# Autodesk Inventor assembly: drivetrain
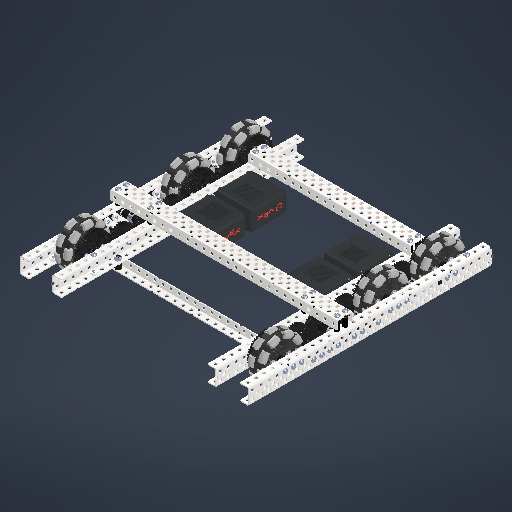
[picture p0: Inventor's stored thumbnail of the model, 512x512]
Saved by Autodesk Inventor 2026.1 (Build 301233000, 233)
## iProperties
Created: 2024-09-29
Part Number: drivetrain
Document SubType Name: Assembly
Designer: Exortions
Author: Exortions
## Documents named in this file (34)
- C:\Users\shimo\OneDrive\Documents\GitHub\cad3284b-2024\second-robot\drivetrain - Copy.iam
- C:\Users\shimo\OneDrive\Documents\GitHub\cad3284b-2024\lib\vex\Structure\C Channel\Aluminum 1x2x1\Alu C 1x2x1x30.ipt
- C:\Users\shimo\OneDrive\Documents\GitHub\cad3284b-2024\lib\vex\Structure\C Channel\Aluminum 1x2x1\Alu C 1x2x1x28.ipt
- C:\Users\shimo\OneDrive\Documents\GitHub\cad3284b-2024\lib\vex\Structure\Hardware\Screw Steel - Star\SScrew Star Smooth .290.ipt
- C:\Users\shimo\OneDrive\Documents\GitHub\cad3284b-2024\lib\vex\Structure\Standoff\Standoff .75.ipt
- C:\Users\shimo\OneDrive\Documents\GitHub\cad3284b-2024\lib\vex\Structure\C Channel\Aluminum 1x2x1\Alu C 1x2x1x26.ipt
- C:\Users\shimo\OneDrive\Documents\GitHub\cad3284b-2024\lib\vex\Structure\C Channel\Aluminum 1x2x1\Alu C 1x2x1x20.ipt
- C:\Users\shimo\OneDrive\Documents\GitHub\cad3284b-2024\lib\vex\Motion\Spacers\Spacer Nylon .375 OD\NSpacer .375 OD x .500.ipt
- C:\Users\shimo\OneDrive\Documents\GitHub\cad3284b-2024\lib\vex\Motion\Spacers\Spacer Nylon .375 OD\NSpacer .375 OD x .375.ipt
- C:\Users\shimo\OneDrive\Documents\GitHub\cad3284b-2024\lib\vex\Structure\Hardware\Nut Alu.ipt
- C:\Users\shimo\OneDrive\Documents\GitHub\cad3284b-2024\lib\vex\Structure\Hardware\Nut Thin Nylock.ipt
- C:\Users\shimo\OneDrive\Documents\GitHub\cad3284b-2024\lib\vex\Structure\Hardware\Screw Steel - Star\SScrew Star Smooth 2.250.ipt
- C:\Users\shimo\OneDrive\Documents\GitHub\cad3284b-2024\second-robot\drivetrain-wheel.iam
- C:\Users\shimo\OneDrive\Documents\GitHub\cad3284b-2024\lib\vex\Structure\Hardware\Nut Keps.ipt
- C:\Users\shimo\OneDrive\Documents\GitHub\cad3284b-2024\lib\vex\Motion\Shaft LS\Bearing Flat.ipt
- C:\Users\shimo\OneDrive\Documents\GitHub\cad3284b-2024\lib\vex\Structure\Hardware\Screw Steel - Star\SScrew Star Smooth .500.ipt
- C:\Users\shimo\OneDrive\Documents\GitHub\cad3284b-2024\lib\vex\Structure\Hardware\Nut Nylon\Nut Nylon - White.ipt
- C:\Users\shimo\OneDrive\Documents\GitHub\cad3284b-2024\lib\vex\Electronics\V5 Motor.ipt
- C:\Users\shimo\OneDrive\Documents\GitHub\cad3284b-2024\lib\vex\Motion\Gears\LS 36T Gear.ipt
- C:\Users\shimo\OneDrive\Documents\GitHub\cad3284b-2024\lib\vex\Motion\Spacers\Washer Teflon\TWasher .375 OD x .06250.ipt
- C:\Users\shimo\OneDrive\Documents\GitHub\cad3284b-2024\lib\vex\Motion\Shaft LS\Shaft Collar ipts\Shaft Collar Set Screw.ipt
- C:\Users\shimo\OneDrive\Documents\GitHub\cad3284b-2024\lib\vex\Motion\Spacers\Spacer Nylon .375 OD\NSpacer .375 OD x .125.ipt
- C:\Users\shimo\OneDrive\Documents\GitHub\cad3284b-2024\lib\vex\Motion\1-Post Bearing Flat Hex Retainer.ipt
- C:\Users\shimo\OneDrive\Documents\GitHub\cad3284b-2024\lib\vex\Structure\C Channel\Aluminum 1x2x1\Alu C 1x2x1x1.ipt
- C:\Users\shimo\OneDrive\Documents\GitHub\cad3284b-2024\lib\vex\Structure\Angle\Aluminum 1x1\Alu Angle 1x1x20.ipt
- C:\Users\shimo\OneDrive\Documents\GitHub\cad3284b-2024\lib\vex\Structure\Hardware\Screw Steel - Star\SScrew Star Smooth .625.ipt
- C:\Users\shimo\OneDrive\Documents\GitHub\cad3284b-2024\lib\vex\Structure\Hardware\Screw Steel - Star.ipt
- C:\Users\shimo\OneDrive\Documents\GitHub\cad3284b-2024\lib\vex\Structure\Standoff.ipt
- C:\Users\shimo\OneDrive\Documents\GitHub\cad3284b-2024\lib\vex\Structure\Hardware\Nut Nylon.ipt
- C:\Users\shimo\OneDrive\Documents\GitHub\cad3284b-2024\lib\vex\Motion\Spacers\Washer Teflon.ipt
- C:\Users\shimo\OneDrive\Documents\GitHub\cad3284b-2024\lib\vex\Motion\Spacers\Spacer Nylon .375 OD.ipt
- C:\Users\shimo\OneDrive\Documents\GitHub\cad3284b-2024\lib\vex\Structure\Standoff\Standoff .50.ipt
- C:\Users\shimo\OneDrive\Documents\GitHub\3284b-highlander-cad\Library\VEX-CAD-Inventor-1.4.2\Structure\C Channel\Aluminum 1x2x1\Alu C 1x2x1x2.ipt
- C:\Users\shimo\OneDrive\Documents\GitHub\3284b-highlander-cad\Library\VEX-CAD-Inventor-1.4.2\Structure\C Channel\Aluminum 1x2x1\Alu C 1x2x1x1.ipt
## Components (224 placed, 27 different names)
1. Alu C 1x2x1x30:1 — Insert:1, Insert:2, Insert:5, Insert:6, Insert:13, Insert:14, Insert:66, Insert:69, Insert:70, Insert:72, Insert:73, Insert:78, Insert:79, Insert:80, Insert:81, Insert:223, Insert:224, Insert:228, Insert:229, Insert:232, Insert:233, Insert:238, Insert:239, Insert:245, Insert:246, Insert:247, Insert:248, Insert:249, Insert:250, Insert:251, Insert:253, Insert:254, Insert:255, Insert:256, Insert:267, Insert:268, Insert:270, Insert:271, Insert:275, Insert:455, Insert:1085
2. Alu C 1x2x1x30:2 — Insert:3, Insert:4, Insert:11, Insert:12, Insert:15, Insert:16, Insert:293, Insert:294, Insert:295, Insert:296, Insert:297, Insert:301, Insert:302, Insert:303, Insert:304, Insert:305, Insert:335, Insert:336, Insert:341, Insert:342, Insert:343, Insert:344, Insert:345, Insert:346, Insert:347, Insert:348, Insert:349, Insert:350, Insert:377, Insert:378, Insert:379, Insert:380, Insert:408, Insert:433, Insert:473
3. Alu C 1x2x1x28:1 — Insert:1, Insert:2, Insert:3, Insert:4, Insert:7, Insert:8, Insert:9, Insert:10, Insert:17, Insert:18, Insert:19, Insert:20, Insert:25, Insert:26, Insert:31, Insert:32, Insert:506, Insert:507, Insert:532, Insert:533, Insert:534, Insert:535
4. SScrew Star Smooth .290:1 — Insert:8
5. SScrew Star Smooth .290:2 — Insert:6
6. SScrew Star Smooth .290:3 — Insert:7
7. SScrew Star Smooth .290:4 — Insert:5
8. SScrew Star Smooth .290:5 — Insert:12
9. SScrew Star Smooth .290:6 — Insert:10
10. SScrew Star Smooth .290:7 — Insert:9
11. SScrew Star Smooth .290:8 — Insert:11
12. Standoff .75:1 — Insert:14
13. Standoff .75:2 — Insert:13
14. Standoff .75:3 — Insert:16
15. Standoff .75:4 — Insert:15
16. Alu C 1x2x1x26:1 — Insert:25, Insert:26, Insert:27, Insert:28, Insert:29, Insert:30, Insert:44, Insert:193, Insert:225, Insert:226, Mate:2, Flush:3, Flush:4, Insert:240, Insert:244, Insert:257, Insert:264, Insert:266, Insert:276, Insert:453, Insert:454, Insert:482, Insert:483, Insert:484, Insert:485, Insert:490, Insert:520, Insert:521, Insert:522, Insert:523, Insert:698, Insert:699, Insert:702, Insert:1034, Insert:1055, Insert:1056, Rigid:4
17. Alu C 1x2x1x26:2 — Insert:19, Insert:20, Insert:21, Insert:22, Insert:23, Insert:24, Insert:46, Mate:1, Flush:1, Flush:2, Insert:325, Insert:327, Insert:331, Insert:332, Insert:369, Insert:375, Insert:409, Insert:431, Insert:432, Insert:451, Insert:475, Insert:476, Insert:479, Insert:480, Insert:481, Insert:491, Insert:512, Insert:513, Insert:514, Insert:515, Insert:704, Insert:1036, Insert:1053, Insert:1054, Rigid:3
18. SScrew Star Smooth .290:9 — Insert:18
19. SScrew Star Smooth .290:10 — Insert:17
20. Standoff .75:5 — Insert:21
21. Standoff .75:6 — Insert:22
22. SScrew Star Smooth .290:11 — Insert:32
23. SScrew Star Smooth .290:12 — Insert:31
24. Standoff .75:7 — Insert:30
25. Standoff .75:8 — Insert:29
26. SScrew Star Smooth .290:13 — Insert:24
27. SScrew Star Smooth .290:14 — Insert:23
28. SScrew Star Smooth .290:15 — Insert:28
29. SScrew Star Smooth .290:16 — Insert:27
30. Alu C 1x2x1x20:1 — Insert:36, Insert:37, Insert:38, Insert:39, Insert:698, Insert:699
31. SScrew Star Smooth .290:17 — Insert:36
32. SScrew Star Smooth .290:18 — Insert:37
33. SScrew Star Smooth .290:19 — Insert:38
34. SScrew Star Smooth .290:20 — Insert:39
35. SScrew Star Smooth .290:22 — Insert:44
36. SScrew Star Smooth .290:24 — Insert:46
37. SScrew Star Smooth 2.250:29 — Insert:66
38. Nut Keps:1 — Insert:71
39. Bearing Flat:1 — Insert:69, Insert:70, Insert:71, Insert:74, Insert:75
40. SScrew Star Smooth .500:30 — Insert:73
41. SScrew Star Smooth .500:31 — Insert:72
42. Nut Nylon - White:1 — Insert:75
43. Nut Nylon - White:2 — Insert:74
44. Bearing Flat:2 — Insert:78, Insert:79, Insert:452
45. Nut Nylon - White:3
46. Nut Nylon - White:4
47. SScrew Star Smooth .500:32 — Insert:81
48. SScrew Star Smooth .500:33 — Insert:80
49. LS 36T Gear:1 — Insert:94, Insert:96
50. TWasher .375 OD x .06250:1 — Insert:94, Insert:453
51. NSpacer .375 OD x .500:11 — Insert:96, Insert:97
52. Shaft Collar Set Screw:1 — Insert:97, Insert:99
53. NSpacer .375 OD x .375:12 — Insert:98, Insert:99
54. TWasher .375 OD x .06250:2 — Insert:98
55. Nut Keps:2
56. Bearing Flat:4 — Insert:247, Insert:248
57. Nut Nylon - White:6
58. Nut Nylon - White:7
59. Bearing Flat:6 — Insert:228, Insert:229
60. Nut Nylon - White:10
61. Nut Nylon - White:11
62. NSpacer .375 OD x .125:13 — Insert:234, Insert:454
63. Nut Keps:5 — Insert:269
64. LS 36T Gear:2
65. TWasher .375 OD x .06250:5 — Insert:244
66. NSpacer .375 OD x .500:16
67. Shaft Collar Set Screw:2
68. NSpacer .375 OD x .375:17
69. TWasher .375 OD x .06250:6
70. LS 36T Gear:3
71. TWasher .375 OD x .06250:7 — Insert:264
72. NSpacer .375 OD x .500:18
73. Shaft Collar Set Screw:3
74. NSpacer .375 OD x .375:19
75. TWasher .375 OD x .06250:8
76. Bearing Flat:10 — Insert:238, Insert:239
77. Nut Nylon - White:18
78. Nut Nylon - White:19
79. Bearing Flat:11 — Insert:253, Insert:254
80. Nut Nylon - White:20
81. Nut Nylon - White:21
82. 1-Post Bearing Flat Hex Retainer:1 — Insert:182, Insert:267, Insert:268, Insert:269
83. Nut Nylon - White:22 — Insert:182
84. SScrew Star Smooth .500:62 — Insert:193
85. SScrew Star Smooth .290:67
86. SScrew Star Smooth .290:69
87. SScrew Star Smooth .290:70
88. Nut Nylon - White:25 — Insert:226
89. Nut Nylon - White:26 — Insert:225
90. Nut Nylon - White:27 — Insert:224
91. Nut Nylon - White:28 — Insert:223
92. Alu C 1x2x1x1:1 — Mate:1, Flush:1, Flush:2, Rigid:1
93. Alu C 1x2x1x1:2 — Mate:2, Flush:3, Flush:4, Rigid:2
94. SScrew Star Smooth .500:72 — Insert:232
95. SScrew Star Smooth .500:73 — Insert:233
96. LS 36T Gear:4 — Insert:234, Insert:237
97. NSpacer .375 OD x .500:31 — Insert:236
98. NSpacer .375 OD x .500:32 — Insert:236, Insert:237
99. SScrew Star Smooth .500:74 — Insert:245
100. SScrew Star Smooth .500:75 — Insert:246
101. SScrew Star Smooth .500:76 — Insert:240
102. SScrew Star Smooth .500:77 — Insert:249
103. SScrew Star Smooth 2.250:78 — Insert:250
104. SScrew Star Smooth .500:79 — Insert:251
105. SScrew Star Smooth .500:80 — Insert:256
106. SScrew Star Smooth .500:81 — Insert:255
107. SScrew Star Smooth .500:82 — Insert:257
108. SScrew Star Smooth .500:84 — Insert:266
109. SScrew Star Smooth .500:85 — Insert:270
110. SScrew Star Smooth 2.250:86 — Insert:271
111. SScrew Star Smooth .290:89
112. Nut Nylon - White:31 — Insert:276
113. SScrew Star Smooth .290:90
114. Nut Nylon - White:32 — Insert:275
115. SScrew Star Smooth 2.250:93 — Insert:295
116. Nut Keps:6
117. Bearing Flat:12 — Insert:293, Insert:294
118. SScrew Star Smooth .500:94 — Insert:297
119. SScrew Star Smooth .500:95 — Insert:296
120. Nut Nylon - White:33
121. Nut Nylon - White:34
122. SScrew Star Smooth 2.250:96 — Insert:305
123. Nut Keps:7
124. Bearing Flat:13 — Insert:301, Insert:302
125. SScrew Star Smooth .500:97 — Insert:303
126. SScrew Star Smooth .500:98 — Insert:304
127. Nut Nylon - White:35
128. Nut Nylon - White:36
129. Nut Keps:9
130. 1-Post Bearing Flat Hex Retainer:2 — Insert:377, Insert:378
131. Nut Nylon - White:39
132. SScrew Star Smooth .500:104 — Insert:325
133. SScrew Star Smooth .500:106 — Insert:327
134. SScrew Star Smooth .500:107 — Insert:331
135. SScrew Star Smooth .500:108 — Insert:332
136. Bearing Flat:16 — Insert:335, Insert:336
137. Nut Nylon - White:41
138. Nut Nylon - White:42
139. SScrew Star Smooth .500:109 — Insert:345
140. SScrew Star Smooth .500:110 — Insert:346
141. Bearing Flat:17 — Insert:341, Insert:342
142. Nut Nylon - White:43
143. Nut Nylon - White:44
144. Bearing Flat:18 — Insert:343, Insert:344, Insert:474
145. Nut Nylon - White:45
146. Nut Nylon - White:46
147. SScrew Star Smooth .500:111 — Insert:347
148. SScrew Star Smooth .500:112 — Insert:348
149. SScrew Star Smooth .500:113 — Insert:349
150. SScrew Star Smooth .500:114 — Insert:350
151. NSpacer .375 OD x .125:45 — Insert:475
152. LS 36T Gear:5
153. NSpacer .375 OD x .500:46
154. NSpacer .375 OD x .500:47
155. LS 36T Gear:6
156. TWasher .375 OD x .06250:9 — Insert:476
157. NSpacer .375 OD x .500:48
158. Shaft Collar Set Screw:4
159. NSpacer .375 OD x .375:49
160. TWasher .375 OD x .06250:10
161. LS 36T Gear:7
162. TWasher .375 OD x .06250:11 — Insert:369
163. NSpacer .375 OD x .500:50
164. Shaft Collar Set Screw:5
165. NSpacer .375 OD x .375:51
166. TWasher .375 OD x .06250:12
167. LS 36T Gear:8
168. TWasher .375 OD x .06250:13 — Insert:375
169. NSpacer .375 OD x .500:52
170. Shaft Collar Set Screw:6
171. NSpacer .375 OD x .375:53
172. TWasher .375 OD x .06250:14
173. SScrew Star Smooth .500:116 — Insert:380
174. SScrew Star Smooth 2.250:117 — Insert:379
175. Nut Nylon - White:47 — Insert:408
176. SScrew Star Smooth .290:124
177. SScrew Star Smooth .290:125
178. Nut Nylon - White:48 — Insert:409
179. SScrew Star Smooth .290:130
180. Nut Nylon - White:50 — Insert:433
181. Nut Nylon - White:51 — Insert:432
182. Nut Nylon - White:53 — Insert:431
183. Alu Angle 1x1x20:1 — Insert:451, Insert:485, Insert:486, Insert:487, Insert:488, Insert:489
184. SScrew Star Smooth 2.250:136 — Insert:455
185. Nut Keps:11 — Insert:452
186. SScrew Star Smooth 2.250:140 — Insert:473
187. Nut Keps:12 — Insert:474
188. drivetrain-wheel:1 [sub-assembly] — Insert:479
189. drivetrain-wheel:2 [sub-assembly] — Insert:480
190. drivetrain-wheel:3 [sub-assembly] — Insert:481
191. drivetrain-wheel:4 [sub-assembly] — Insert:484
192. drivetrain-wheel:5 [sub-assembly] — Insert:483
193. drivetrain-wheel:6 [sub-assembly] — Insert:482
194. NSpacer .375 OD x .375:73 — Insert:487
195. NSpacer .375 OD x .375:74 — Insert:486
196. SScrew Star Smooth .625:144 — Insert:489
197. SScrew Star Smooth .625:145 — Insert:488
198. Nut Thin Nylock:11 — Insert:490
199. Nut Thin Nylock:12 — Insert:491
200. Nut Alu:5 — Insert:507
201. Nut Alu:6 — Insert:506
202. V5 Motor:9 — Insert:512, Insert:513
203. V5 Motor:10 — Insert:514, Insert:515
204. V5 Motor:12 — Insert:520, Insert:521
205. V5 Motor:13 — Insert:522, Insert:523
206. Nut Alu:7 — Insert:532
207. Nut Alu:8 — Insert:533
208. Nut Alu:9 — Insert:534
209. Nut Alu:10 — Insert:535
210. SScrew Star Smooth .290:200 — Insert:702
211. SScrew Star Smooth .290:201 — Insert:704
212. Nut Nylon - White:69 — Insert:1034
213. SScrew Star Smooth .290:281
214. Nut Nylon - White:70 — Insert:1036
215. SScrew Star Smooth .290:282
216. Standoff .50:44 — Insert:1055
217. Standoff .50:45 — Insert:1056
218. Standoff .50:46 — Insert:1054
219. Standoff .50:47 — Insert:1053
220. Nut Thin Nylock:56 — Insert:1085
221. Alu C 1x2x1x2:1 — Rigid:4
222. Alu C 1x2x1x2:2 — Rigid:3
223. Alu C 1x2x1x1:4 — Rigid:1
224. Alu C 1x2x1x1:5 — Rigid:2
## Relationships (240: Insert 230, Flush 4, WeldJoint 4, Mate 2)
- Insert:1 (19.05 mm): Alu C 1x2x1x30:1 ↔ Alu C 1x2x1x28:1
- Insert:2 (19.05 mm): Alu C 1x2x1x30:1 ↔ Alu C 1x2x1x28:1
- Insert:3 (19.05 mm): Alu C 1x2x1x30:2 ↔ Alu C 1x2x1x28:1
- Insert:4 (19.05 mm): Alu C 1x2x1x30:2 ↔ Alu C 1x2x1x28:1
- Insert:5: Alu C 1x2x1x30:1 ↔ SScrew Star Smooth .290:4
- Insert:6: Alu C 1x2x1x30:1 ↔ SScrew Star Smooth .290:2
- Insert:7: Alu C 1x2x1x28:1 ↔ SScrew Star Smooth .290:3
- Insert:8: Alu C 1x2x1x28:1 ↔ SScrew Star Smooth .290:1
- Insert:9: Alu C 1x2x1x28:1 ↔ SScrew Star Smooth .290:7
- Insert:10: Alu C 1x2x1x28:1 ↔ SScrew Star Smooth .290:6
- Insert:11: Alu C 1x2x1x30:2 ↔ SScrew Star Smooth .290:8
- Insert:12: Alu C 1x2x1x30:2 ↔ SScrew Star Smooth .290:5
- Insert:13: Alu C 1x2x1x30:1 ↔ Standoff .75:2
- Insert:14: Alu C 1x2x1x30:1 ↔ Standoff .75:1
- Insert:15: Alu C 1x2x1x30:2 ↔ Standoff .75:4
- Insert:16: Alu C 1x2x1x30:2 ↔ Standoff .75:3
- Insert:17: Alu C 1x2x1x28:1 ↔ SScrew Star Smooth .290:10
- Insert:18: Alu C 1x2x1x28:1 ↔ SScrew Star Smooth .290:9
- Insert:19 (19.05 mm): Alu C 1x2x1x28:1 ↔ Alu C 1x2x1x26:2
- Insert:20 (19.05 mm): Alu C 1x2x1x28:1 ↔ Alu C 1x2x1x26:2
- Insert:21: Alu C 1x2x1x26:2 ↔ Standoff .75:5
- Insert:22: Alu C 1x2x1x26:2 ↔ Standoff .75:6
- Insert:23: Alu C 1x2x1x26:2 ↔ SScrew Star Smooth .290:14
- Insert:24: Alu C 1x2x1x26:2 ↔ SScrew Star Smooth .290:13
- Insert:25 (19.05 mm): Alu C 1x2x1x28:1 ↔ Alu C 1x2x1x26:1
- Insert:26 (19.05 mm): Alu C 1x2x1x28:1 ↔ Alu C 1x2x1x26:1
- Insert:27: Alu C 1x2x1x26:1 ↔ SScrew Star Smooth .290:16
- Insert:28: Alu C 1x2x1x26:1 ↔ SScrew Star Smooth .290:15
- Insert:29: Alu C 1x2x1x26:1 ↔ Standoff .75:8
- Insert:30: Alu C 1x2x1x26:1 ↔ Standoff .75:7
- Insert:31: Alu C 1x2x1x28:1 ↔ SScrew Star Smooth .290:12
- Insert:32: Alu C 1x2x1x28:1 ↔ SScrew Star Smooth .290:11
- Insert:36: Alu C 1x2x1x20:1 ↔ SScrew Star Smooth .290:17
- Insert:37: Alu C 1x2x1x20:1 ↔ SScrew Star Smooth .290:18
- Insert:38: Alu C 1x2x1x20:1 ↔ SScrew Star Smooth .290:19
- Insert:39: Alu C 1x2x1x20:1 ↔ SScrew Star Smooth .290:20
- Insert:44: Alu C 1x2x1x26:1 ↔ SScrew Star Smooth .290:22
- Insert:46: Alu C 1x2x1x26:2 ↔ SScrew Star Smooth .290:24
- Insert:66: Alu C 1x2x1x30:1 ↔ SScrew Star Smooth 2.250:29
- Insert:69: Alu C 1x2x1x30:1 ↔ Bearing Flat:1
- Insert:70: Alu C 1x2x1x30:1 ↔ Bearing Flat:1
- Insert:71: Nut Keps:1 ↔ Bearing Flat:1
- Insert:72: Alu C 1x2x1x30:1 ↔ SScrew Star Smooth .500:31
- Insert:73: Alu C 1x2x1x30:1 ↔ SScrew Star Smooth .500:30
- Insert:74: Bearing Flat:1 ↔ Nut Nylon - White:2
- Insert:75: Bearing Flat:1 ↔ Nut Nylon - White:1
- [Insert]: Bearing Flat:2 ↔ Nut Nylon - White:4
- [Insert]: Bearing Flat:2 ↔ Nut Nylon - White:3
- Insert:78: Alu C 1x2x1x30:1 ↔ Bearing Flat:2
- Insert:79: Alu C 1x2x1x30:1 ↔ Bearing Flat:2
- Insert:80: Alu C 1x2x1x30:1 ↔ SScrew Star Smooth .500:33
- Insert:81: Alu C 1x2x1x30:1 ↔ SScrew Star Smooth .500:32
- Insert:94: LS 36T Gear:1 ↔ TWasher .375 OD x .06250:1
- Insert:96: LS 36T Gear:1 ↔ NSpacer .375 OD x .500:11
- Insert:97: NSpacer .375 OD x .500:11 ↔ Shaft Collar Set Screw:1
- Insert:98: NSpacer .375 OD x .375:12 ↔ TWasher .375 OD x .06250:2
- Insert:99: Shaft Collar Set Screw:1 ↔ NSpacer .375 OD x .375:12
- [Insert]: Nut Keps:2 ↔ Bearing Flat:4
- [Insert]: Bearing Flat:4 ↔ Nut Nylon - White:7
- [Insert]: Bearing Flat:4 ↔ Nut Nylon - White:6
- [Insert]: Bearing Flat:6 ↔ Nut Nylon - White:11
- [Insert]: Bearing Flat:6 ↔ Nut Nylon - White:10
- [Insert]: LS 36T Gear:2 ↔ TWasher .375 OD x .06250:5
- [Insert]: LS 36T Gear:2 ↔ NSpacer .375 OD x .500:16
- [Insert]: NSpacer .375 OD x .500:16 ↔ Shaft Collar Set Screw:2
- [Insert]: NSpacer .375 OD x .375:17 ↔ TWasher .375 OD x .06250:6
- [Insert]: Shaft Collar Set Screw:2 ↔ NSpacer .375 OD x .375:17
- [Insert]: LS 36T Gear:3 ↔ TWasher .375 OD x .06250:7
- [Insert]: LS 36T Gear:3 ↔ NSpacer .375 OD x .500:18
- [Insert]: NSpacer .375 OD x .500:18 ↔ Shaft Collar Set Screw:3
- [Insert]: NSpacer .375 OD x .375:19 ↔ TWasher .375 OD x .06250:8
- [Insert]: Shaft Collar Set Screw:3 ↔ NSpacer .375 OD x .375:19
- [Insert]: Bearing Flat:10 ↔ Nut Nylon - White:19
- [Insert]: Bearing Flat:10 ↔ Nut Nylon - White:18
- [Insert]: Bearing Flat:11 ↔ Nut Nylon - White:21
- [Insert]: Bearing Flat:11 ↔ Nut Nylon - White:20
- Insert:182: 1-Post Bearing Flat Hex Retainer:1 ↔ Nut Nylon - White:22
- Insert:193: Alu C 1x2x1x26:1 ↔ SScrew Star Smooth .500:62
- Insert:223: Alu C 1x2x1x30:1 ↔ Nut Nylon - White:28
- Insert:224: Alu C 1x2x1x30:1 ↔ Nut Nylon - White:27
- Insert:225: Alu C 1x2x1x26:1 ↔ Nut Nylon - White:26
- Insert:226: Alu C 1x2x1x26:1 ↔ Nut Nylon - White:25
- Mate:1: Alu C 1x2x1x26:2 ↔ Alu C 1x2x1x1:1
- Flush:1: Alu C 1x2x1x26:2 ↔ Alu C 1x2x1x1:1
- Flush:2: Alu C 1x2x1x26:2 ↔ Alu C 1x2x1x1:1
- Mate:2: Alu C 1x2x1x26:1 ↔ Alu C 1x2x1x1:2
- Flush:3: Alu C 1x2x1x26:1 ↔ Alu C 1x2x1x1:2
- Flush:4: Alu C 1x2x1x26:1 ↔ Alu C 1x2x1x1:2
- Insert:228: Alu C 1x2x1x30:1 ↔ Bearing Flat:6
- Insert:229: Alu C 1x2x1x30:1 ↔ Bearing Flat:6
- Insert:232: Alu C 1x2x1x30:1 ↔ SScrew Star Smooth .500:72
- Insert:233: Alu C 1x2x1x30:1 ↔ SScrew Star Smooth .500:73
- Insert:234: NSpacer .375 OD x .125:13 ↔ LS 36T Gear:4
- Insert:236: NSpacer .375 OD x .500:31 ↔ NSpacer .375 OD x .500:32
- Insert:237: LS 36T Gear:4 ↔ NSpacer .375 OD x .500:32
- Insert:238: Alu C 1x2x1x30:1 ↔ Bearing Flat:10
- Insert:239: Alu C 1x2x1x30:1 ↔ Bearing Flat:10
- Insert:240: Alu C 1x2x1x26:1 ↔ SScrew Star Smooth .500:76
- Insert:244: Alu C 1x2x1x26:1 ↔ TWasher .375 OD x .06250:5
- Insert:245: Alu C 1x2x1x30:1 ↔ SScrew Star Smooth .500:74
- Insert:246: Alu C 1x2x1x30:1 ↔ SScrew Star Smooth .500:75
- Insert:247: Alu C 1x2x1x30:1 ↔ Bearing Flat:4
- Insert:248: Alu C 1x2x1x30:1 ↔ Bearing Flat:4
- Insert:249: Alu C 1x2x1x30:1 ↔ SScrew Star Smooth .500:77
- Insert:250: Alu C 1x2x1x30:1 ↔ SScrew Star Smooth 2.250:78
- Insert:251: Alu C 1x2x1x30:1 ↔ SScrew Star Smooth .500:79
- Insert:253: Alu C 1x2x1x30:1 ↔ Bearing Flat:11
- Insert:254: Alu C 1x2x1x30:1 ↔ Bearing Flat:11
- Insert:255: Alu C 1x2x1x30:1 ↔ SScrew Star Smooth .500:81
- Insert:256: Alu C 1x2x1x30:1 ↔ SScrew Star Smooth .500:80
- Insert:257: Alu C 1x2x1x26:1 ↔ SScrew Star Smooth .500:82
- Insert:264: Alu C 1x2x1x26:1 ↔ TWasher .375 OD x .06250:7
- Insert:266: Alu C 1x2x1x26:1 ↔ SScrew Star Smooth .500:84
- Insert:267: Alu C 1x2x1x30:1 ↔ 1-Post Bearing Flat Hex Retainer:1
- Insert:268: Alu C 1x2x1x30:1 ↔ 1-Post Bearing Flat Hex Retainer:1
- Insert:269: Nut Keps:5 ↔ 1-Post Bearing Flat Hex Retainer:1
- Insert:270: Alu C 1x2x1x30:1 ↔ SScrew Star Smooth .500:85
- Insert:271: Alu C 1x2x1x30:1 ↔ SScrew Star Smooth 2.250:86
- Insert:275: Alu C 1x2x1x30:1 ↔ Nut Nylon - White:32
- Insert:276: Alu C 1x2x1x26:1 ↔ Nut Nylon - White:31
- [Insert]: Nut Keps:6 ↔ Bearing Flat:12
- [Insert]: Bearing Flat:12 ↔ Nut Nylon - White:34
- [Insert]: Bearing Flat:12 ↔ Nut Nylon - White:33
- Insert:293: Alu C 1x2x1x30:2 ↔ Bearing Flat:12
- Insert:294: Alu C 1x2x1x30:2 ↔ Bearing Flat:12
- Insert:295: Alu C 1x2x1x30:2 ↔ SScrew Star Smooth 2.250:93
- Insert:296: Alu C 1x2x1x30:2 ↔ SScrew Star Smooth .500:95
- Insert:297: Alu C 1x2x1x30:2 ↔ SScrew Star Smooth .500:94
- [Insert]: Nut Keps:7 ↔ Bearing Flat:13
- [Insert]: Bearing Flat:13 ↔ Nut Nylon - White:36
- [Insert]: Bearing Flat:13 ↔ Nut Nylon - White:35
- Insert:301: Alu C 1x2x1x30:2 ↔ Bearing Flat:13
- Insert:302: Alu C 1x2x1x30:2 ↔ Bearing Flat:13
- Insert:303: Alu C 1x2x1x30:2 ↔ SScrew Star Smooth .500:97
- Insert:304: Alu C 1x2x1x30:2 ↔ SScrew Star Smooth .500:98
- Insert:305: Alu C 1x2x1x30:2 ↔ SScrew Star Smooth 2.250:96
- [Insert]: 1-Post Bearing Flat Hex Retainer:2 ↔ Nut Nylon - White:39
- [Insert]: Nut Keps:9 ↔ 1-Post Bearing Flat Hex Retainer:2
- Insert:325: Alu C 1x2x1x26:2 ↔ SScrew Star Smooth .500:104
- Insert:327: Alu C 1x2x1x26:2 ↔ SScrew Star Smooth .500:106
- Insert:331: Alu C 1x2x1x26:2 ↔ SScrew Star Smooth .500:107
- Insert:332: Alu C 1x2x1x26:2 ↔ SScrew Star Smooth .500:108
- [Insert]: Bearing Flat:16 ↔ Nut Nylon - White:42
- [Insert]: Bearing Flat:16 ↔ Nut Nylon - White:41
- Insert:335: Alu C 1x2x1x30:2 ↔ Bearing Flat:16
- Insert:336: Alu C 1x2x1x30:2 ↔ Bearing Flat:16
- [Insert]: Bearing Flat:17 ↔ Nut Nylon - White:44
- [Insert]: Bearing Flat:17 ↔ Nut Nylon - White:43
- [Insert]: Bearing Flat:18 ↔ Nut Nylon - White:46
- [Insert]: Bearing Flat:18 ↔ Nut Nylon - White:45
- Insert:341: Alu C 1x2x1x30:2 ↔ Bearing Flat:17
- Insert:342: Alu C 1x2x1x30:2 ↔ Bearing Flat:17
- Insert:343: Alu C 1x2x1x30:2 ↔ Bearing Flat:18
- Insert:344: Alu C 1x2x1x30:2 ↔ Bearing Flat:18
- Insert:345: Alu C 1x2x1x30:2 ↔ SScrew Star Smooth .500:109
- Insert:346: Alu C 1x2x1x30:2 ↔ SScrew Star Smooth .500:110
- Insert:347: Alu C 1x2x1x30:2 ↔ SScrew Star Smooth .500:111
- Insert:348: Alu C 1x2x1x30:2 ↔ SScrew Star Smooth .500:112
- Insert:349: Alu C 1x2x1x30:2 ↔ SScrew Star Smooth .500:113
- Insert:350: Alu C 1x2x1x30:2 ↔ SScrew Star Smooth .500:114
- [Insert]: NSpacer .375 OD x .125:45 ↔ LS 36T Gear:5
- [Insert]: NSpacer .375 OD x .500:46 ↔ NSpacer .375 OD x .500:47
- [Insert]: LS 36T Gear:5 ↔ NSpacer .375 OD x .500:47
- [Insert]: LS 36T Gear:6 ↔ TWasher .375 OD x .06250:9
- [Insert]: LS 36T Gear:6 ↔ NSpacer .375 OD x .500:48
- [Insert]: NSpacer .375 OD x .500:48 ↔ Shaft Collar Set Screw:4
- [Insert]: NSpacer .375 OD x .375:49 ↔ TWasher .375 OD x .06250:10
- [Insert]: Shaft Collar Set Screw:4 ↔ NSpacer .375 OD x .375:49
- [Insert]: LS 36T Gear:7 ↔ TWasher .375 OD x .06250:11
- [Insert]: LS 36T Gear:7 ↔ NSpacer .375 OD x .500:50
- [Insert]: NSpacer .375 OD x .500:50 ↔ Shaft Collar Set Screw:5
- [Insert]: NSpacer .375 OD x .375:51 ↔ TWasher .375 OD x .06250:12
- [Insert]: Shaft Collar Set Screw:5 ↔ NSpacer .375 OD x .375:51
- Insert:369: Alu C 1x2x1x26:2 ↔ TWasher .375 OD x .06250:11
- [Insert]: LS 36T Gear:8 ↔ TWasher .375 OD x .06250:13
- [Insert]: LS 36T Gear:8 ↔ NSpacer .375 OD x .500:52
- [Insert]: NSpacer .375 OD x .500:52 ↔ Shaft Collar Set Screw:6
- [Insert]: NSpacer .375 OD x .375:53 ↔ TWasher .375 OD x .06250:14
- [Insert]: Shaft Collar Set Screw:6 ↔ NSpacer .375 OD x .375:53
- Insert:375: Alu C 1x2x1x26:2 ↔ TWasher .375 OD x .06250:13
- Insert:377: Alu C 1x2x1x30:2 ↔ 1-Post Bearing Flat Hex Retainer:2
- Insert:378: Alu C 1x2x1x30:2 ↔ 1-Post Bearing Flat Hex Retainer:2
- Insert:379: Alu C 1x2x1x30:2 ↔ SScrew Star Smooth 2.250:117
- Insert:380: Alu C 1x2x1x30:2 ↔ SScrew Star Smooth .500:116
- Insert:408: Alu C 1x2x1x30:2 ↔ Nut Nylon - White:47
- Insert:409: Alu C 1x2x1x26:2 ↔ Nut Nylon - White:48
- Insert:431: Alu C 1x2x1x26:2 ↔ Nut Nylon - White:53
- Insert:432: Alu C 1x2x1x26:2 ↔ Nut Nylon - White:51
- Insert:433: Alu C 1x2x1x30:2 ↔ Nut Nylon - White:50
- Insert:451 (9.525 mm): Alu C 1x2x1x26:2 ↔ Alu Angle 1x1x20:1
- Insert:452: Bearing Flat:2 ↔ Nut Keps:11
- Insert:453: Alu C 1x2x1x26:1 ↔ TWasher .375 OD x .06250:1
- Insert:454: Alu C 1x2x1x26:1 ↔ NSpacer .375 OD x .125:13
- Insert:455: Alu C 1x2x1x30:1 ↔ SScrew Star Smooth 2.250:136
- Insert:473: Alu C 1x2x1x30:2 ↔ SScrew Star Smooth 2.250:140
- Insert:474: Bearing Flat:18 ↔ Nut Keps:12
- Insert:475: Alu C 1x2x1x26:2 ↔ NSpacer .375 OD x .125:45
- Insert:476: Alu C 1x2x1x26:2 ↔ TWasher .375 OD x .06250:9
- Insert:479: Alu C 1x2x1x26:2 ↔ drivetrain-wheel:1
- Insert:480: Alu C 1x2x1x26:2 ↔ drivetrain-wheel:2
- Insert:481: Alu C 1x2x1x26:2 ↔ drivetrain-wheel:3
- Insert:482: Alu C 1x2x1x26:1 ↔ drivetrain-wheel:6
- Insert:483: Alu C 1x2x1x26:1 ↔ drivetrain-wheel:5
- Insert:484: Alu C 1x2x1x26:1 ↔ drivetrain-wheel:4
- Insert:485 (9.525 mm): Alu C 1x2x1x26:1 ↔ Alu Angle 1x1x20:1
- Insert:486: Alu Angle 1x1x20:1 ↔ NSpacer .375 OD x .375:74
- Insert:487: Alu Angle 1x1x20:1 ↔ NSpacer .375 OD x .375:73
- Insert:488: Alu Angle 1x1x20:1 ↔ SScrew Star Smooth .625:145
- Insert:489: Alu Angle 1x1x20:1 ↔ SScrew Star Smooth .625:144
- Insert:490: Alu C 1x2x1x26:1 ↔ Nut Thin Nylock:11
- Insert:491: Alu C 1x2x1x26:2 ↔ Nut Thin Nylock:12
- Insert:506: Alu C 1x2x1x28:1 ↔ Nut Alu:6
- Insert:507: Alu C 1x2x1x28:1 ↔ Nut Alu:5
- Insert:512: Alu C 1x2x1x26:2 ↔ V5 Motor:9
- Insert:513: Alu C 1x2x1x26:2 ↔ V5 Motor:9
- Insert:514: Alu C 1x2x1x26:2 ↔ V5 Motor:10
- Insert:515: Alu C 1x2x1x26:2 ↔ V5 Motor:10
- Insert:520: Alu C 1x2x1x26:1 ↔ V5 Motor:12
- Insert:521: Alu C 1x2x1x26:1 ↔ V5 Motor:12
- Insert:522: Alu C 1x2x1x26:1 ↔ V5 Motor:13
- Insert:523: Alu C 1x2x1x26:1 ↔ V5 Motor:13
- Insert:532: Alu C 1x2x1x28:1 ↔ Nut Alu:7
- Insert:533: Alu C 1x2x1x28:1 ↔ Nut Alu:8
- Insert:534: Alu C 1x2x1x28:1 ↔ Nut Alu:9
- Insert:535: Alu C 1x2x1x28:1 ↔ Nut Alu:10
- Insert:698 (12.7 mm): Alu C 1x2x1x26:1 ↔ Alu C 1x2x1x20:1
- Insert:699 (12.7 mm): Alu C 1x2x1x26:1 ↔ Alu C 1x2x1x20:1
- Insert:702: Alu C 1x2x1x26:1 ↔ SScrew Star Smooth .290:200
- Insert:704: Alu C 1x2x1x26:2 ↔ SScrew Star Smooth .290:201
- Insert:1034: Alu C 1x2x1x26:1 ↔ Nut Nylon - White:69
- Insert:1036: Alu C 1x2x1x26:2 ↔ Nut Nylon - White:70
- Insert:1053: Alu C 1x2x1x26:2 ↔ Standoff .50:47
- Insert:1054: Alu C 1x2x1x26:2 ↔ Standoff .50:46
- Insert:1055: Alu C 1x2x1x26:1 ↔ Standoff .50:44
- Insert:1056: Alu C 1x2x1x26:1 ↔ Standoff .50:45
- Insert:1085: Alu C 1x2x1x30:1 ↔ Nut Thin Nylock:56
- Rigid:1 [WeldJoint]: Alu C 1x2x1x1:1 ↔ Alu C 1x2x1x1:4
- Rigid:2 [WeldJoint]: Alu C 1x2x1x1:2 ↔ Alu C 1x2x1x1:5
- Rigid:3 [WeldJoint]: Alu C 1x2x1x26:2 ↔ Alu C 1x2x1x2:2
- Rigid:4 [WeldJoint]: Alu C 1x2x1x26:1 ↔ Alu C 1x2x1x2:1
## Named parameters: d96_d94 = 0 mm, d97_d95 = 0 mm, d125_d91 = 0 mm, d126_d94 = 0 mm, d127_d95 = 0 mm, d149_d94 = 0 mm, d150_d95 = 0 mm, d191_d118 = 0 mm, d192_d121 = 0 mm, d193_d122 = 0 mm, d194_d123 = 0 mm, d195_d124 = 0 mm, d196_d118 = 0 mm, d197_d121 = 0 mm, d198_d122 = 0 mm, d199_d123 = 0 mm, d200_d124 = 0 mm, d203_d96_d94 = 0 mm, d204_d97_d95 = 0 mm, d209_d96_d94 = 0 mm, d210_d97_d95 = 0 mm, d362_d91 = 0 mm, d363_d94 = 0 mm, d364_d95 = 0 mm, d370_d91 = 0 mm, d371_d94 = 0 mm, d372_d95 = 0 mm, d386_d341 = 0 mm, d387_d217 = 0 mm, d405_d203_d96_d94 = 0 mm, d406_d204_d97_d95 = 0 mm, d409_d405_d203_d96_d94 = 0 mm, d410_d406_d204_d97_d95 = 0 mm, d411_d405_d203_d96_d94 = 0 mm, d412_d406_d204_d97_d95 = 0 mm, d425_d299 = 0 mm, d426_d306 = 0 mm, d427_d307 = 0 mm, d429_d118 = 0 mm, d430_d121 = 0 mm, d431_d122 = 0 mm, d432_d123 = 0 mm, d433_d124 = 0 mm, d436_d191_d118 = 0 mm, d437_d192_d121 = 0 mm, d438_d193_d122 = 0 mm, d439_d194_d123 = 0 mm, d440_d195_d124 = 0 mm, d442_d196_d118 = 0 mm, d443_d197_d121 = 0 mm, d444_d198_d122 = 0 mm, d445_d199_d123 = 0 mm, d446_d200_d124 = 0 mm
